# Autodesk Inventor assembly: Weapon Assembly
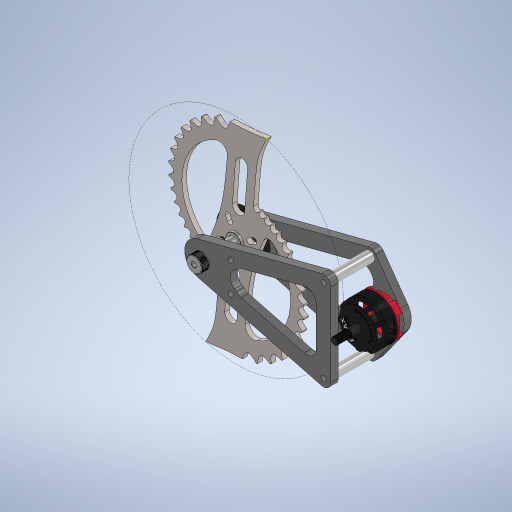
[picture p0: Inventor's stored thumbnail of the model, 512x512]
Saved by Autodesk Inventor 2023.1 (Build 271208000, 208)
## iProperties
Created: 2022-08-25
Part Number: Weapon Assembly
Document SubType Name: Assembly
Designer: Nathan Cai
Mass: 140.161 g
Surface Area: 396.844 cm^2
Volume: 43.633 cm^3
Density: 3.21227 g/cm^3
Author: Nathan Cai
## Documents named in this file (8)
- E:\Documents\Inventor\3rd Lawelle - V0.1\Weapon Assembly.iam
- E:\Documents\Inventor\3rd Lawelle - V0.1\Arm (Motor).ipt
- E:\Documents\Inventor\3rd Lawelle - V0.1\Arm (Brace).ipt
- E:\Documents\Inventor\3rd Lawelle - V0.1\EMAX motor\MOTOR EMAX RS2205.iam
- E:\Documents\Inventor\3rd Lawelle - V0.1\Spacer 1in.ipt
- E:\Documents\Inventor\3rd Lawelle - V0.1\92981A120_Alloy Steel Shoulder Screws.ipt
- E:\Documents\Inventor\3rd Lawelle - V0.1\90237A120_High-Strength Steel Nylon-Insert Locknuts.ipt
- E:\Documents\Inventor\3rd Lawelle - V0.1\Blade Assembly.iam
## Components (8 placed, 7 different names)
1. Arm (Motor):1 — Mate:1, Mate:2, Mate:3, Mate:4, Mate:5, Mate:8, Mate:9, Mate:13
2. Arm (Brace):1 — Mate:1, Mate:2, Mate:6, Mate:7, Mate:10, Mate:11, Mate:12, Mate:16
3. MOTOR EMAX RS2205:1 [sub-assembly] — Mate:3, Mate:4, Mate:5
4. Spacer 1in:1 — Mate:6, Mate:9, Mate:10
5. Spacer 1in:2 — Mate:7, Mate:8
6. 92981A120_Alloy Steel Shoulder Screws:1 — Mate:11, Mate:12, Mate:14, Mate:15
7. 90237A120_High-Strength Steel Nylon-Insert Locknuts:1 — Mate:13, Mate:14
8. Blade Assembly:1 [sub-assembly] — Mate:15, Mate:16
## Relationships (16: Mate 16)
- Mate:1: Arm (Motor):1 ↔ Arm (Brace):1
- Mate:2: Arm (Motor):1 ↔ Arm (Brace):1
- Mate:3: Arm (Motor):1 ↔ MOTOR EMAX RS2205:1
- Mate:4: Arm (Motor):1 ↔ MOTOR EMAX RS2205:1
- Mate:5: Arm (Motor):1 ↔ MOTOR EMAX RS2205:1
- Mate:6: Arm (Brace):1 ↔ Spacer 1in:1
- Mate:7: Arm (Brace):1 ↔ Spacer 1in:2
- Mate:8: Arm (Motor):1 ↔ Spacer 1in:2
- Mate:9: Arm (Motor):1 ↔ Spacer 1in:1
- Mate:10: Arm (Brace):1 ↔ Spacer 1in:1
- Mate:11: Arm (Brace):1 ↔ 92981A120_Alloy Steel Shoulder Screws:1
- Mate:12: Arm (Brace):1 ↔ 92981A120_Alloy Steel Shoulder Screws:1
- Mate:13: Arm (Motor):1 ↔ 90237A120_High-Strength Steel Nylon-Insert Locknuts:1
- Mate:14: 92981A120_Alloy Steel Shoulder Screws:1 ↔ 90237A120_High-Strength Steel Nylon-Insert Locknuts:1
- Mate:15: 92981A120_Alloy Steel Shoulder Screws:1 ↔ Blade Assembly:1
- Mate:16: Arm (Brace):1 ↔ Blade Assembly:1
